# Autodesk Inventor assembly: Assembly3
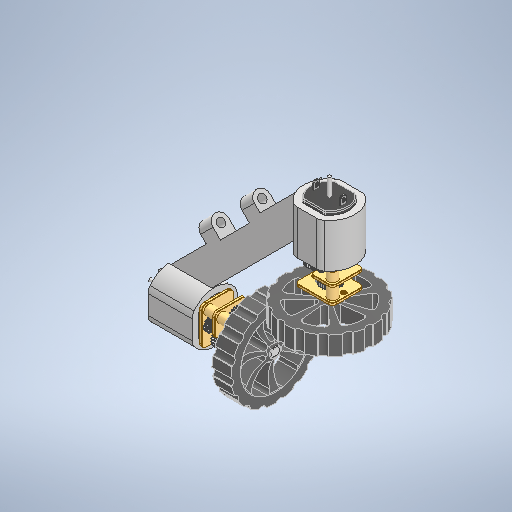
[picture p0: Inventor's stored thumbnail of the model, 512x512]
Saved by Autodesk Inventor 2025.1 (Build 291241000, 241)
## iProperties
Created: 2026-05-05
Part Number: Assembly3
Document SubType Name: Assembly
Designer: User
Author: User
## Documents named in this file (5)
- D:\One Drive\OneDrive - Politeknik Sultan Salahuddin Abdul Aziz Shah\Documents\Inventor\RobosotPSA\Assembly3.iam
- Dribbler_Type1.iam
- D:\One Drive\OneDrive - Politeknik Sultan Salahuddin Abdul Aziz Shah\Documents\Inventor\RobosotPSA\wheel v7\wheel v7\Drib_v1.ipt
- D:\One Drive\OneDrive - Politeknik Sultan Salahuddin Abdul Aziz Shah\Documents\Inventor\RobosotPSA\N20 Mini Micro Metall Gear Motor DC 3-6-12V v1\N20 Mini Micro Metall Gear Motor DC 3-6-12V v1\N20 Mini Micro Me.ipt
- D:\One Drive\OneDrive - Politeknik Sultan Salahuddin Abdul Aziz Shah\Documents\Inventor\RobosotPSA\wheel v7\wheel v7\wheel v7.ipt
## Components (5 placed, 3 different names)
1. Drib_v1:1 — Flush:1, Mate:1, Mate:2, Mate:3, Mate:4, Flush:2
2. N20 Mini Micro Me:1 — Flush:1, Mate:1, Mate:2, Mate:5, Flush:3
3. N20 Mini Micro Me:2 — Mate:3, Mate:4, Flush:2, Flush:4, Mate:6
4. wheel v7:1 — Flush:4, Mate:6
5. wheel v7:2 — Mate:5, Flush:3
## Relationships (10: Mate 6, Flush 4)
- Flush:1 (1 mm): Drib_v1:1 ↔ N20 Mini Micro Me:1
- Mate:1 (0.1 mm): Drib_v1:1 ↔ N20 Mini Micro Me:1
- Mate:2: Drib_v1:1 ↔ N20 Mini Micro Me:1
- Mate:3 (0.1 mm): Drib_v1:1 ↔ N20 Mini Micro Me:2
- Mate:4: Drib_v1:1 ↔ N20 Mini Micro Me:2
- Flush:2 (-1 mm): Drib_v1:1 ↔ N20 Mini Micro Me:2
- Mate:5: N20 Mini Micro Me:1 ↔ wheel v7:2
- Flush:3: N20 Mini Micro Me:1 ↔ wheel v7:2
- Flush:4: N20 Mini Micro Me:2 ↔ wheel v7:1
- Mate:6: N20 Mini Micro Me:2 ↔ wheel v7:1
